# Autodesk Inventor assembly: 动力传输1
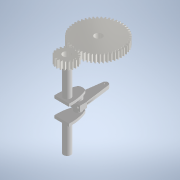
[picture p0: Inventor's stored thumbnail of the model, 180x180]
Saved by Autodesk Inventor 2022 (Build 260153000, 153)
## iProperties
Created: 2023-02-21
Part Number: 动力传输1
Document SubType Name: Assembly
Designer: 李承轩
Author: 李承轩
## Documents named in this file (5)
- D:\Person products\发动机模型\动力传输1.iam
- D:\Person products\发动机模型\动力传输1\设计加速器\正齿轮4.iam
- D:\Person products\发动机模型\曲轴.ipt
- D:\Person products\发动机模型\连接下环.ipt
- D:\Person products\发动机模型\连杆.ipt
## Components (4 placed, 4 different names)
1. 正齿轮:2 [sub-assembly] — 表面齐平:1
2. 曲轴:1 — 表面齐平:1, 表面齐平:2
3. 连接下环:1 — 表面齐平:2, 表面齐平:3
4. 连杆:1 — 表面齐平:3
## Relationships (3: Flush 3)
- 表面齐平:1 [Flush]: 正齿轮:2 ↔ 曲轴:1
- 表面齐平:2 [Flush]: 曲轴:1 ↔ 连接下环:1
- 表面齐平:3 [Flush]: 连接下环:1 ↔ 连杆:1
